# Autodesk Inventor assembly: Upperarm
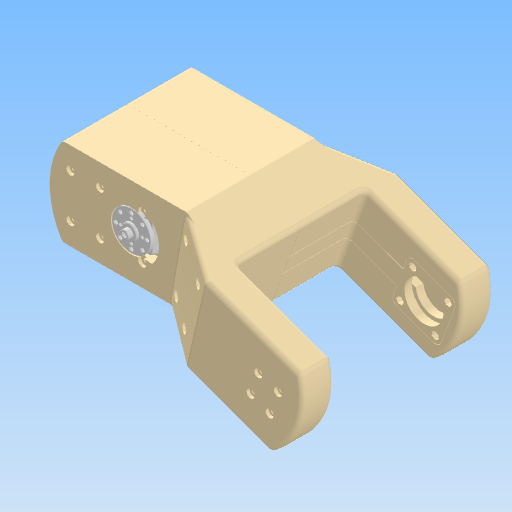
[picture p0: Inventor's stored thumbnail of the model, 512x512]
Saved by Autodesk Inventor 2021 (Build 250183000, 183)
## iProperties
Created: 2020-02-11
Part Number: Upperarm
Document SubType Name: Assembly
Designer: JochenAlt
Author: JochenAlt
## Documents named in this file (3)
- C:\Users\Jochen Alt\Documents\Daten\Projects\MiniBot\CAD\Upperarm.iam
- C:\Users\Jochen Alt\Documents\Daten\Projects\MiniBot\CAD\Upperarm.ipt
- C:\Users\Jochen Alt\Documents\Daten\Projects\MiniBot\CAD\extern\Herkulex\Herkulex DRS-040x.ipt
## Components (3 placed, 2 different names)
1. Upperarm:1 — Winkel:1, Passend:3, Fluchtend:2
2. Herkulex DRS-040x:1 — Passend:1, Passend:2, Fluchtend:1, Winkel:1
3. Herkulex DRS-040x:2 — Passend:1, Passend:2, Fluchtend:1, Passend:3, Fluchtend:2
## Relationships (6: Mate 3, Flush 2, Angle 1)
- Passend:1 [Mate]: Herkulex DRS-040x:1 ↔ Herkulex DRS-040x:2
- Passend:2 [Mate] (0.2 mm): Herkulex DRS-040x:1 ↔ Herkulex DRS-040x:2
- Fluchtend:1 [Flush]: Herkulex DRS-040x:1 ↔ Herkulex DRS-040x:2
- Winkel:1 [Angle] (-90 deg): Upperarm:1 ↔ Herkulex DRS-040x:1
- Passend:3 [Mate]: Upperarm:1 ↔ Herkulex DRS-040x:2
- Fluchtend:2 [Flush]: Upperarm:1 ↔ Herkulex DRS-040x:2
